# Autodesk Inventor assembly: Assy_flame_back
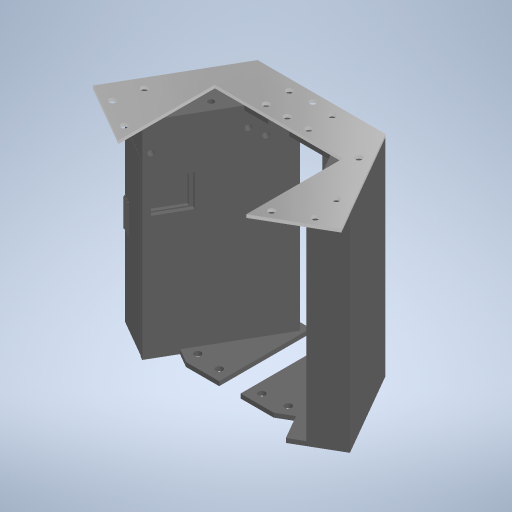
[picture p0: Inventor's stored thumbnail of the model, 512x512]
Saved by Autodesk Inventor 2024.1 (Build 281209000, 209)
## iProperties
Created: 2025-04-23
Part Number: Assy_flame_back
Document SubType Name: Assembly
Designer: hibik
Author: hibik
## Documents named in this file (7)
- C:\Users\hibik\Documents\Robomech\RESCUE\ORCA\hard\flame_back\Assy_flame_back.iam
- C:\Users\hibik\Documents\Robomech\RESCUE\ORCA\hard\flame_back\flame_back.ipt
- C:\Users\hibik\Documents\Robomech\RESCUE\ORCA\hard\flame_back\flame_upper_back.ipt
- C:\Users\hibik\Documents\Robomech\RESCUE\ORCA\hard\flame_back\battery_holder_spring.ipt
- C:\Users\hibik\Documents\Robomech\RESCUE\ORCA\hard\flame_back\battery_holder_cover.ipt
- C:\Users\hibik\Documents\Robomech\RESCUE\ORCA\hard\flame_back\battery_case.ipt
- C:\Users\hibik\Documents\Robomech\RESCUE\ORCA\hard\flame_back\battery_case_cover.ipt
## Components (6 placed, 6 different names)
1. flame_back:1 — 挿入:1, 挿入:2, 挿入:3, 挿入:4, 挿入:5, メイト:1, メイト:2
2. flame_upper_back:1 — 挿入:1, 挿入:2
3. battery_holder_spring:1 — 挿入:3
4. battery_holder_cover:1 — 挿入:4, 挿入:5
5. battery_case:1 — メイト:1, メイト:2, メイト:3, メイト:4, メイト:5
6. battery_case_cover:1 — メイト:3, メイト:4, メイト:5
## Relationships (10: Insert 5, Mate 5)
- 挿入:1 [Insert]: flame_back:1 ↔ flame_upper_back:1
- 挿入:2 [Insert]: flame_back:1 ↔ flame_upper_back:1
- 挿入:3 [Insert]: flame_back:1 ↔ battery_holder_spring:1
- 挿入:4 [Insert]: flame_back:1 ↔ battery_holder_cover:1
- 挿入:5 [Insert]: flame_back:1 ↔ battery_holder_cover:1
- メイト:1 [Mate]: flame_back:1 ↔ battery_case:1
- メイト:2 [Mate]: flame_back:1 ↔ battery_case:1
- メイト:3 [Mate]: battery_case:1 ↔ battery_case_cover:1
- メイト:4 [Mate]: battery_case:1 ↔ battery_case_cover:1
- メイト:5 [Mate]: battery_case:1 ↔ battery_case_cover:1
